# Autodesk Inventor assembly: Ensamblaje1
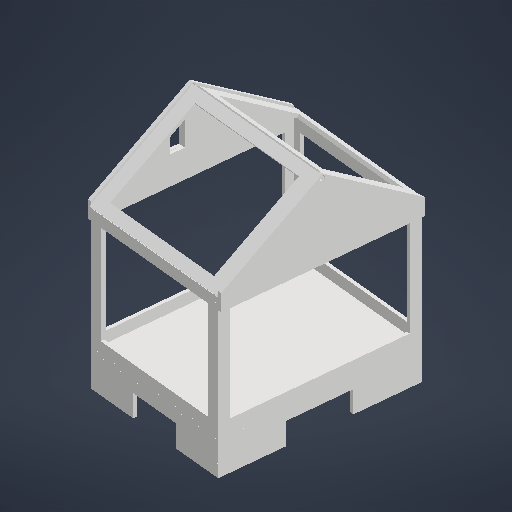
[picture p0: Inventor's stored thumbnail of the model, 512x512]
Saved by Autodesk Inventor 2026.1 (Build 301233020, 233B)
## iProperties
Created: 2026-05-06
Part Number: Ensamblaje1
Document SubType Name: Assembly
Designer: OlmesTech
Author: OlmesTech
## Documents named in this file (11)
- C:\Users\OlmesTech\OneDrive\Escritorio\Ensamblaje1.iam
- C:\Users\OlmesTech\OneDrive\Escritorio\Pieza2.ipt
- C:\Users\OlmesTech\OneDrive\Escritorio\Pieza1.ipt
- C:\Users\OlmesTech\OneDrive\Escritorio\Pieza3.ipt
- C:\Users\OlmesTech\OneDrive\Escritorio\Pieza4.ipt
- C:\Users\OlmesTech\OneDrive\Escritorio\Pieza5.ipt
- C:\Users\OlmesTech\OneDrive\Escritorio\Pieza7.ipt
- C:\Users\OlmesTech\OneDrive\Escritorio\Pieza10.ipt
- C:\Users\OlmesTech\OneDrive\Escritorio\Pieza11.ipt
- C:\Users\OlmesTech\OneDrive\Escritorio\Pieza8.ipt
- C:\Users\OlmesTech\OneDrive\Escritorio\Pieza6.ipt
## Components (13 placed, 10 different names)
1. Pieza2:1 — Nivelación:1, Coincidencia:2, Nivelación:3
2. Pieza1:1 — Nivelación:1, Coincidencia:2, Nivelación:2, Nivelación:4
3. Pieza2:2 — Nivelación:2, Coincidencia:11
4. Pieza1:2 — Nivelación:3
5. Pieza3:1 — Nivelación:4, Nivelación:5, Nivelación:6, Coincidencia:7, Coincidencia:9, Coincidencia:10
6. Pieza6:1 — Nivelación:5, Nivelación:12, Coincidencia:12
7. Pieza4:2 — Nivelación:6, Coincidencia:7, Nivelación:7, Coincidencia:8, Nivelación:8, Nivelación:9, Nivelación:11
8. Pieza5:1 — Nivelación:7, Coincidencia:8, Coincidencia:9, Coincidencia:13
9. Pieza5:2 — Coincidencia:10, Nivelación:8, Coincidencia:11
10. Pieza7:1 — Nivelación:9
11. Pieza10:1 — Nivelación:11
12. Pieza11:1 — Nivelación:12
13. Pieza8:1 — Coincidencia:12, Coincidencia:13
## Relationships (19: Flush 11, Mate 8)
- Nivelación:1 [Flush]: Pieza2:1 ↔ Pieza1:1
- Coincidencia:2 [Mate]: Pieza2:1 ↔ Pieza1:1
- Nivelación:2 [Flush]: Pieza1:1 ↔ Pieza2:2
- Nivelación:3 [Flush]: Pieza2:1 ↔ Pieza1:2
- Nivelación:4 [Flush]: Pieza1:1 ↔ Pieza3:1
- Nivelación:5 [Flush]: Pieza3:1 ↔ Pieza6:1
- Nivelación:6 [Flush]: Pieza3:1 ↔ Pieza4:2
- Coincidencia:7 [Mate]: Pieza3:1 ↔ Pieza4:2
- Nivelación:7 [Flush]: Pieza4:2 ↔ Pieza5:1
- Coincidencia:8 [Mate]: Pieza4:2 ↔ Pieza5:1
- Coincidencia:9 [Mate]: Pieza3:1 ↔ Pieza5:1
- Coincidencia:10 [Mate]: Pieza3:1 ↔ Pieza5:2
- Nivelación:8 [Flush]: Pieza4:2 ↔ Pieza5:2
- Coincidencia:11 [Mate]: Pieza2:2 ↔ Pieza5:2
- Nivelación:9 [Flush]: Pieza4:2 ↔ Pieza7:1
- Nivelación:11 [Flush]: Pieza4:2 ↔ Pieza10:1
- Nivelación:12 [Flush]: Pieza6:1 ↔ Pieza11:1
- Coincidencia:12 [Mate]: Pieza6:1 ↔ Pieza8:1
- Coincidencia:13 [Mate]: Pieza5:1 ↔ Pieza8:1
